# Autodesk Inventor assembly: 132
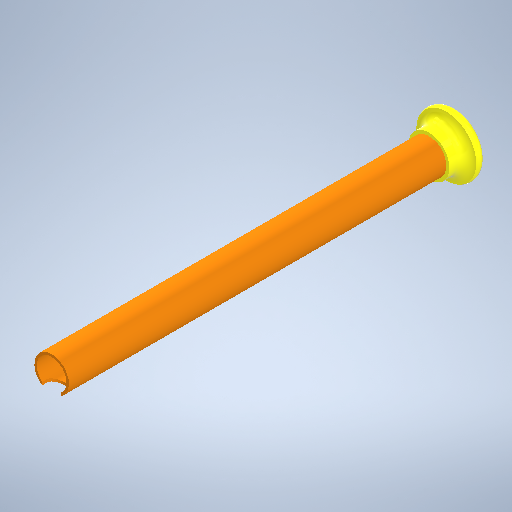
[picture p0: Inventor's stored thumbnail of the model, 512x512]
Saved by Autodesk Inventor 2025.1 (Build 291241000, 241)
## iProperties
Created: 2024-08-01
Part Number: 132
Document SubType Name: Assembly
Designer: ffogue
Author: ffogue
## Documents named in this file (3)
- C:\Projkete - Übungen\Freedom\132.iam
- C:\Projkete - Übungen\Freedom\132 part 1.ipt
- C:\Projkete - Übungen\Freedom\132 part 2.ipt
## Components (2 placed, 2 different names)
1. 132 part 1:1 — Mate:1, Insert:1
2. 132 part 2:1 — Mate:1, Insert:1
## Relationships (2: Mate 1, Insert 1)
- Mate:1: 132 part 1:1 ↔ 132 part 2:1
- Insert:1 (-20 mm): 132 part 1:1 ↔ 132 part 2:1
